# Autodesk Inventor assembly: stand
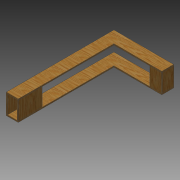
[picture p0: Inventor's stored thumbnail of the model, 180x180]
Saved by Autodesk Inventor 2013 (Build 170138000, 138)
## iProperties
Created: 2014-10-20
Part Number: stand
Document SubType Name: Assembly
Designer: Masta
Author: Masta
## Documents named in this file (5)
- D:\DrOctopus\3D model\stand.iam
- D:\DrOctopus\3D model\stand_plate1.ipt
- D:\DrOctopus\3D model\stand_plate2.ipt
- D:\DrOctopus\3D model\stand_plate3.ipt
- D:\DrOctopus\3D model\stand_plate4.ipt
## Components (6 placed, 4 different names)
1. stand_plate1:1 — Mate:1, Flush:1, Flush:2, Mate:2, Flush:3
2. stand_plate1:2 — Mate:4, Flush:4, Flush:5, Mate:5, Mate:6, Flush:6, Flush:7, Flush:8, Flush:9
3. stand_plate2:1 — Mate:1, Flush:1, Flush:2, Mate:3, Mate:4, Flush:4, Flush:5
4. stand_plate3:1 — Mate:2, Flush:3, Mate:3
5. stand_plate4:1 — Mate:5, Flush:7, Flush:9
6. stand_plate4:2 — Mate:6, Flush:6, Flush:8
## Relationships (15: Flush 9, Mate 6)
- Mate:1: stand_plate1:1 ↔ stand_plate2:1
- Flush:1: stand_plate1:1 ↔ stand_plate2:1
- Flush:2: stand_plate1:1 ↔ stand_plate2:1
- Mate:2: stand_plate1:1 ↔ stand_plate3:1
- Flush:3: stand_plate1:1 ↔ stand_plate3:1
- Mate:3: stand_plate2:1 ↔ stand_plate3:1
- Mate:4: stand_plate1:2 ↔ stand_plate2:1
- Flush:4: stand_plate1:2 ↔ stand_plate2:1
- Flush:5: stand_plate1:2 ↔ stand_plate2:1
- Mate:5: stand_plate1:2 ↔ stand_plate4:1
- Mate:6: stand_plate1:2 ↔ stand_plate4:2
- Flush:6: stand_plate1:2 ↔ stand_plate4:2
- Flush:7: stand_plate1:2 ↔ stand_plate4:1
- Flush:8: stand_plate1:2 ↔ stand_plate4:2
- Flush:9: stand_plate1:2 ↔ stand_plate4:1
